# Autodesk Inventor assembly: Draft_02_Combined
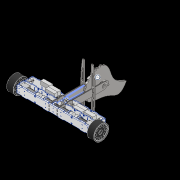
[picture p0: Inventor's stored thumbnail of the model, 180x180]
Saved by Autodesk Inventor 2021 (Build 250183000, 183)
## iProperties
Created: 2021-03-10
Part Number: Draft_02_Combined
Document SubType Name: Assembly
Designer: M3rob
Mass: 102210 g
Surface Area: 54892 cm^2
Volume: 35052.9 cm^3
Density: 2.91588 g/cm^3
Author: M3rob
## Documents named in this file (38)
- C:\Users\Esketitttttt\Documents\GrabCAD\FireBird 250 Pound Gaming Machine\Drafts\FrameDrafts\Draft_Wide01\Draft_Wide01_Combined.iam
- C:\Users\Esketitttttt\Documents\GrabCAD\FireBird 250 Pound Gaming Machine\Drafts\FrameDrafts\Draft_Wide01\NeckFrame_03.ipt
- C:\Users\Esketitttttt\Documents\GrabCAD\FireBird 250 Pound Gaming Machine\Drafts\FrameDrafts\Draft_Wide01\FrontWallFrame_03.ipt
- C:\Users\Esketitttttt\Documents\GrabCAD\FireBird 250 Pound Gaming Machine\Drafts\FrameDrafts\Draft_Wide01\BackWallFrame_03.ipt
- C:\Users\Esketitttttt\Documents\GrabCAD\FireBird 250 Pound Gaming Machine\Drafts\FrameDrafts\Draft_Wide01\SmallSideFrame_03.ipt
- C:\Users\Esketitttttt\Documents\GrabCAD\FireBird 250 Pound Gaming Machine\Drafts\FrameDrafts\Draft_Wide01\DriveSideFrame_03.ipt
- C:\Users\Esketitttttt\Documents\GrabCAD\FireBird 250 Pound Gaming Machine\Drafts\FrameDrafts\Draft_Wide01\6524K421_FRICTION TORQUE LIMITER.ipt
- C:\Users\Esketitttttt\Documents\GrabCAD\FireBird 250 Pound Gaming Machine\Drafts\FrameDrafts\Draft_Wide01\MotorMountingPlates.ipt
- C:\Users\Esketitttttt\Documents\GrabCAD\FireBird 250 Pound Gaming Machine\Drafts\FrameDrafts\Draft_Wide01\MotorMockup.ipt
- C:\Users\Esketitttttt\Documents\GrabCAD\FireBird 250 Pound Gaming Machine\Drafts\FrameDrafts\Draft_Wide01\GearboxMockup.ipt
- C:\Users\M3rob\Documents\Inventor\Content Center Files\R2021\en-US\AS 2465(2)\AS 2465 - 3_8 x 1 1_4  UNC.ipt
- C:\Users\M3rob\Documents\Inventor\Content Center Files\R2021\en-US\AS 2465(1)\AS 2465 - 3_8  UNC(1).ipt
- C:\Users\M3rob\Documents\Inventor\Content Center Files\R2021\en-US\U UNC 2603(1)\Unbrako - 8 x 1 1_4 - 32 - 1.25 - Unbrako.ipt
- C:\Users\M3rob\Documents\Inventor\Content Center Files\R2021\en-US\U UNC 2603(1)\Unbrako - 5_16 x 1 3_4 - 18 - 1.75 - Unbrako.ipt
- C:\Users\Esketitttttt\Documents\GrabCAD\FireBird 250 Pound Gaming Machine\Drafts\FrameDrafts\Draft_Wide01\Chain Drive1.iam
- C:\Users\Esketitttttt\Documents\GrabCAD\FireBird 250 Pound Gaming Machine\Drafts\FrameDrafts\Draft_Wide01\Chain Drive2.iam
- C:\Users\Esketitttttt\Documents\GrabCAD\FireBird 250 Pound Gaming Machine\Drafts\FrameDrafts\Draft_Wide01\Chain Drive3.iam
- C:\Users\Esketitttttt\Documents\GrabCAD\FireBird 250 Pound Gaming Machine\Drafts\FrameDrafts\Draft_Wide01\Bearing1.iam
- C:\Users\Esketitttttt\Documents\GrabCAD\FireBird 250 Pound Gaming Machine\Drafts\FrameDrafts\Draft_Wide01\Shaft4.ipt
- C:\Users\Esketitttttt\Documents\GrabCAD\FireBird 250 Pound Gaming Machine\Drafts\FrameDrafts\Draft_Wide01\WeaponDraft02.ipt
- C:\Users\Esketitttttt\Documents\GrabCAD\FireBird 250 Pound Gaming Machine\Drafts\FrameDrafts\Draft_Wide01\TopBottomUHMW.ipt
- C:\Users\Esketitttttt\Documents\GrabCAD\FireBird 250 Pound Gaming Machine\Drafts\FrameDrafts\Draft_Wide01\FrontWallUHMW.ipt
- C:\Users\Esketitttttt\Documents\GrabCAD\FireBird 250 Pound Gaming Machine\Drafts\FrameDrafts\Draft_Wide01\Bearing3.iam
- C:\Users\Esketitttttt\Documents\GrabCAD\FireBird 250 Pound Gaming Machine\Drafts\FrameDrafts\Draft_Wide01\Shaft5.ipt
- C:\Users\Esketitttttt\Documents\GrabCAD\FireBird 250 Pound Gaming Machine\Drafts\FrameDrafts\Draft_Wide01\SmallFrontWallUHMW.ipt
- C:\Users\M3rob\Documents\Inventor\Content Center Files\R2021\en-US\AS 2465(2)\AS 2465 - 3_8 x 1 1_2  UNC.ipt
- C:\Users\M3rob\Documents\Inventor\Content Center Files\R2021\en-US\ANSI B18.2.2(09)\ANSI B18.2.2 - 3_8 - 16(2).ipt
- C:\Users\M3rob\Documents\Inventor\Content Center Files\R2021\en-US\AS 2465(2)\AS 2465 - 3_8 x 2  UNC.ipt
- C:\Users\M3rob\Documents\Inventor\Content Center Files\R2021\en-US\AS 2465(2)\AS 2465 - 3_8 x 2 1_2  UNC.ipt
- C:\Users\Esketitttttt\Documents\GrabCAD\FireBird 250 Pound Gaming Machine\Drafts\FrameDrafts\Draft_Wide01\MotorCircularClamp.ipt
- C:\Users\Esketitttttt\Documents\GrabCAD\FireBird 250 Pound Gaming Machine\Drafts\FrameDrafts\Draft_Wide01\MotorClampUhmw.ipt
- C:\Users\Esketitttttt\Documents\GrabCAD\FireBird 250 Pound Gaming Machine\Drafts\FrameDrafts\Draft_Wide01\MockupWheel.ipt
- C:\Users\Esketitttttt\Documents\GrabCAD\FireBird 250 Pound Gaming Machine\Drafts\FrameDrafts\Draft_Wide01\WheelHubMockup.ipt
- C:\Users\Esketitttttt\Documents\GrabCAD\FireBird 250 Pound Gaming Machine\Drafts\FrameDrafts\Draft_Wide01\ThiccUpright.ipt
- C:\Users\Esketitttttt\Documents\GrabCAD\FireBird 250 Pound Gaming Machine\Drafts\FrameDrafts\Draft_Wide01\Battery Mockup.ipt
- C:\Users\Esketitttttt\Documents\GrabCAD\FireBird 250 Pound Gaming Machine\Drafts\FrameDrafts\Draft_Wide01\EscMockup.ipt
- C:\Users\Esketitttttt\Documents\GrabCAD\FireBird 250 Pound Gaming Machine\Drafts\FrameDrafts\Draft_Wide01\Whyachi_MS-2PowerSwitch.ipt
- C:\Users\Esketitttttt\Documents\GrabCAD\FireBird 250 Pound Gaming Machine\Drafts\FrameDrafts\Draft_Wide01\MidWallFrame_03.ipt
## Components (214 placed, 33 different names)
1. NeckFrame_03:1 — Mate:1, Mate:3, Mate:4, Mate:5, Mate:12, Mate:14, Mate:17, Mate:18, Mate:40, Mate:41, Mate:42, Mate:47, Mate:71, Mate:73, Mate:75, Mate:77, Mate:98, Mate:99, Mate:104, Flush:4, Mate:125, Flush:18, Mate:260, Mate:384, Mate:385, Mate:386
2. NeckFrame_03:2 — Mate:1, Mate:6, Mate:7, Mate:8, Mate:9, Mate:10, Mate:11, Mate:19, Mate:43, Mate:44, Mate:45, Mate:46, Mate:87, Mate:89, Mate:91, Mate:93, Mate:103, Mate:105, Flush:3, Mate:110, Mate:111, Mate:119, Mate:123, Mate:124, Mate:381, Mate:382, Mate:383, Flush:46, Mate:420
3. MidWallFrame_03:1 — Mate:9, Mate:10, Mate:11, Mate:20, Mate:21, Mate:22
4. FrontWallFrame_03:2 — Mate:6, Mate:7, Mate:8, Flush:10, Flush:11, Mate:165, Mate:167, Mate:169, Mate:171, Mate:173, Mate:175, Mate:177, Mate:179, Mate:181, Mate:183, Mate:185, Mate:187, Mate:189, Mate:191, Mate:193, Mate:195, Mate:229, Mate:231, Mate:233, Mate:235, Mate:237, Mate:239, Mate:241, Mate:243, Mate:245, Mate:247, Mate:249, Mate:251, Mate:253, Mate:255, Mate:257, Mate:259, Mate:276, Mate:278, Mate:280, Mate:282, Mate:284, Mate:286
5. FrontWallFrame_03:3 — Mate:3, Mate:4, Mate:5, Mate:23, Mate:24, Mate:25, Mate:300, Mate:302, Mate:304, Mate:306, Mate:308, Mate:310
6. MidWallFrame_03:2 — Mate:12, Mate:14, Mate:260, Mate:410
7. BackWallFrame_03:1 — Mate:17, Mate:18, Mate:19, Mate:37, Mate:38, Mate:348, Mate:350, Mate:352, Mate:354, Mate:356, Mate:358, Mate:360, Mate:362, Mate:364, Mate:366, Mate:368, Mate:370, Mate:372, Mate:374, Mate:418, Mate:419, Flush:45, Flush:46, Mate:420, Flush:47
8. SmallSideFrame_03:1 — Mate:20, Mate:21, Mate:22, Flush:9, Flush:13, Mate:128
9. SmallSideFrame_03:2 — Mate:23, Mate:24, Mate:25, Mate:261, Mate:316, Mate:318
10. DriveSideFrame_03:1 — Insert:9, Insert:10, Insert:11, Insert:12, Mate:378, Mate:379, Mate:380, Insert:27, Mate:418, Mate:419, Flush:45
11. DriveSideFrame_03:2 — Mate:37, Mate:38, Mate:57, Mate:59, Insert:13, Insert:14, Insert:15, Insert:16, Mate:377, Insert:29, Flush:47
12. 6524K421_FRICTION TORQUE LIMITER:1 — Mate:94, Flush:2, Mate:96
13. 6524K421_FRICTION TORQUE LIMITER:2 — Mate:95, Flush:1, Mate:97
14. Chain Drive:1 [sub-assembly]
15. Chain Drive:2 [sub-assembly] — Mate:112, Mate:375
16. Chain Drive:3 [sub-assembly]
17. Bearing:1 [sub-assembly] — Mate:103, Mate:104
18. Bearing:2 [sub-assembly] — Mate:105, Flush:3
19. Shaft:1 — Mate:112, Mate:113, Angle:1
20. WeaponDraft02:1 — Mate:110, Mate:111
21. TopBottomUHMW:1 — Flush:11, Flush:13, Mate:196, Mate:197, Mate:198, Mate:199, Mate:200, Mate:201, Mate:202, Mate:203, Mate:204, Mate:205, Mate:206, Mate:207, Mate:208, Mate:209, Mate:210, Mate:211, Mate:212, Mate:213, Mate:214, Mate:215, Mate:216, Mate:217, Mate:218, Mate:219, Mate:220, Mate:221, Mate:222, Mate:223, Mate:224, Mate:225, Mate:226, Mate:227, Mate:228, Mate:230, Mate:232, Mate:234, Mate:236, Mate:238, Mate:240, Mate:242, Mate:244, Mate:246, Mate:248, Mate:250, Mate:252, Mate:254, Mate:256, Mate:258
22. TopBottomUHMW:2 — Flush:9, Flush:10, Mate:118, Flush:14, Flush:19, Mate:132, Mate:133, Mate:134, Mate:135, Mate:136, Mate:137, Mate:138, Mate:139, Mate:140, Mate:141, Mate:142, Mate:143, Mate:144, Mate:145, Mate:146, Mate:147, Mate:148, Mate:149, Mate:150, Mate:151, Mate:152, Mate:153, Mate:154, Mate:155, Mate:156, Mate:157, Mate:158, Mate:159, Mate:160, Mate:161, Mate:162, Mate:163, Mate:164, Mate:166, Mate:168, Mate:170, Mate:172, Mate:174, Mate:176, Mate:178, Mate:180, Mate:182, Mate:184, Mate:186, Mate:188, Mate:190, Mate:192, Mate:194, Flush:23
23. FrontWallUHMW:1 — Mate:118, Flush:14, Mate:119, Mate:129, Mate:263, Mate:264, Mate:265, Mate:266, Mate:267, Mate:268, Mate:269, Mate:270, Mate:271, Mate:272, Mate:273, Mate:274, Mate:275, Mate:277, Mate:279, Mate:281, Mate:283, Mate:285
24. Bearing:3 [sub-assembly] — Mate:123, Mate:124
25. SmallFrontWallUHMW:1 — Mate:261, Flush:23, Mate:311, Mate:312, Mate:313, Mate:314, Mate:315, Mate:317
26. SmallFrontWallUHMW:2 — Mate:128, Mate:129, Flush:19
27. ThiccUpright:1 — Mate:381, Mate:382, Mate:383
28. ThiccUpright:2 — Mate:384, Mate:385, Mate:386
29. MotorMountingPlates:1 — Mate:40, Mate:41, Mate:42, Mate:49, Mate:62, Mate:63, Mate:64, Mate:65, Mate:66, Mate:67, Mate:68, Mate:69, Mate:70, Mate:72, Mate:74, Mate:76, Insert:5, Insert:6, Insert:7, Insert:8, Mate:96
30. MotorMountingPlates:2 — Mate:43, Mate:44, Mate:45, Mate:50, Mate:78, Mate:79, Mate:80, Mate:81, Mate:82, Mate:83, Mate:84, Mate:85, Mate:86, Mate:88, Mate:90, Mate:92, Insert:1, Insert:2, Insert:3, Insert:4, Mate:97
31. MotorMockup:1 — Mate:46, Mate:50, Mate:95, Flush:1, Insert:21
32. MotorMockup:2 — Mate:47, Mate:49, Mate:94, Flush:2, Insert:24
33. MotorMockup:3 — Mate:60, Mate:61, Insert:23
34. MotorMockup:4 — Insert:22, Insert:25
35. GearboxMockup:1 — Mate:57, Mate:59, Mate:60, Mate:61, Mate:377, Angle:4
36. GearboxMockup:2 — Mate:378, Mate:379, Mate:380, Insert:25, Angle:3
37. AS 2465 - Inch 3/8 x 1 1/4  UNC:1 — Mate:62, Mate:63
38. AS 2465 - Inch 3/8  UNC:1 — Mate:70, Mate:71
39. AS 2465 - Inch 3/8 x 1 1/4  UNC:2 — Mate:64, Mate:65
40. AS 2465 - Inch 3/8 x 1 1/4  UNC:3 — Mate:66, Mate:67
41. AS 2465 - Inch 3/8 x 1 1/4  UNC:4 — Mate:68, Mate:69
42. AS 2465 - Inch 3/8  UNC:2 — Mate:72, Mate:73
43. AS 2465 - Inch 3/8  UNC:3 — Mate:74, Mate:75
44. AS 2465 - Inch 3/8  UNC:4 — Mate:76, Mate:77
45. AS 2465 - Inch 3/8 x 1 1/4  UNC:5 — Mate:78, Mate:79
46. AS 2465 - Inch 3/8  UNC:5 — Mate:86, Mate:87
47. AS 2465 - Inch 3/8 x 1 1/4  UNC:6 — Mate:80, Mate:81
48. AS 2465 - Inch 3/8 x 1 1/4  UNC:7 — Mate:82, Mate:83
49. AS 2465 - Inch 3/8 x 1 1/4  UNC:8 — Mate:84, Mate:85
50. AS 2465 - Inch 3/8  UNC:6 — Mate:88, Mate:89
51. AS 2465 - Inch 3/8  UNC:7 — Mate:90, Mate:91
52. AS 2465 - Inch 3/8  UNC:8 — Mate:92, Mate:93
53. Unbrako UNC Hex Socket Cap - Inch 8 x 1 1/4:1 — Insert:1
54. Unbrako UNC Hex Socket Cap - Inch 8 x 1 1/4:2 — Insert:2
55. Unbrako UNC Hex Socket Cap - Inch 8 x 1 1/4:3 — Insert:3
56. Unbrako UNC Hex Socket Cap - Inch 8 x 1 1/4:4 — Insert:4
57. Unbrako UNC Hex Socket Cap - Inch 8 x 1 1/4:5 — Insert:5
58. Unbrako UNC Hex Socket Cap - Inch 8 x 1 1/4:6 — Insert:6
59. Unbrako UNC Hex Socket Cap - Inch 8 x 1 1/4:7 — Insert:7
60. Unbrako UNC Hex Socket Cap - Inch 8 x 1 1/4:8 — Insert:8
61. Unbrako UNC Hex Socket Cap - Inch 5/16 x 1 3/4:1 — Insert:9
62. Unbrako UNC Hex Socket Cap - Inch 5/16 x 1 3/4:2 — Insert:10
63. Unbrako UNC Hex Socket Cap - Inch 5/16 x 1 3/4:3 — Insert:11
64. Unbrako UNC Hex Socket Cap - Inch 5/16 x 1 3/4:4 — Insert:12
65. Unbrako UNC Hex Socket Cap - Inch 5/16 x 1 3/4:5 — Insert:13
66. Unbrako UNC Hex Socket Cap - Inch 5/16 x 1 3/4:6 — Insert:14
67. Unbrako UNC Hex Socket Cap - Inch 5/16 x 1 3/4:7 — Insert:15
68. Unbrako UNC Hex Socket Cap - Inch 5/16 x 1 3/4:8 — Insert:16
69. Bearing:4 [sub-assembly] — Mate:125, Flush:18
70. Shaft:1 — Mate:375, Mate:376, Angle:2
71. AS 2465 - Inch 3/8 x 1 1/2  UNC:1 — Mate:132, Mate:133
72. Hex Nut - Inch 3/8 - 16:1 — Mate:164, Mate:165
73. AS 2465 - Inch 3/8 x 1 1/2  UNC:2 — Mate:134, Mate:135
74. AS 2465 - Inch 3/8 x 1 1/2  UNC:3 — Mate:136, Mate:137
75. AS 2465 - Inch 3/8 x 1 1/2  UNC:4 — Mate:138, Mate:139
76. AS 2465 - Inch 3/8 x 1 1/2  UNC:5 — Mate:140, Mate:141
77. AS 2465 - Inch 3/8 x 1 1/2  UNC:6 — Mate:142, Mate:143
78. AS 2465 - Inch 3/8 x 1 1/2  UNC:7 — Mate:144, Mate:145
79. AS 2465 - Inch 3/8 x 1 1/2  UNC:8 — Mate:146, Mate:147
80. AS 2465 - Inch 3/8 x 1 1/2  UNC:9 — Mate:148, Mate:149
81. AS 2465 - Inch 3/8 x 1 1/2  UNC:10 — Mate:150, Mate:151
82. AS 2465 - Inch 3/8 x 1 1/2  UNC:11 — Mate:152, Mate:153
83. AS 2465 - Inch 3/8 x 1 1/2  UNC:12 — Mate:154, Mate:155
84. AS 2465 - Inch 3/8 x 1 1/2  UNC:13 — Mate:156, Mate:157
85. AS 2465 - Inch 3/8 x 1 1/2  UNC:14 — Mate:158, Mate:159
86. AS 2465 - Inch 3/8 x 1 1/2  UNC:15 — Mate:160, Mate:161
87. AS 2465 - Inch 3/8 x 1 1/2  UNC:16 — Mate:162, Mate:163
88. Hex Nut - Inch 3/8 - 16:2 — Mate:166, Mate:167
89. Hex Nut - Inch 3/8 - 16:3 — Mate:168, Mate:169
90. Hex Nut - Inch 3/8 - 16:4 — Mate:170, Mate:171
91. Hex Nut - Inch 3/8 - 16:5 — Mate:172, Mate:173
92. Hex Nut - Inch 3/8 - 16:6 — Mate:174, Mate:175
93. Hex Nut - Inch 3/8 - 16:7 — Mate:176, Mate:177
94. Hex Nut - Inch 3/8 - 16:8 — Mate:178, Mate:179
95. Hex Nut - Inch 3/8 - 16:9 — Mate:180, Mate:181
96. Hex Nut - Inch 3/8 - 16:10 — Mate:182, Mate:183
97. Hex Nut - Inch 3/8 - 16:11 — Mate:184, Mate:185
98. Hex Nut - Inch 3/8 - 16:12 — Mate:186, Mate:187
99. Hex Nut - Inch 3/8 - 16:13 — Mate:188, Mate:189
100. Hex Nut - Inch 3/8 - 16:14 — Mate:190, Mate:191
101. Hex Nut - Inch 3/8 - 16:15 — Mate:192, Mate:193
102. Hex Nut - Inch 3/8 - 16:16 — Mate:194, Mate:195
103. AS 2465 - Inch 3/8 x 1 1/2  UNC:17 — Mate:196, Mate:197
104. Hex Nut - Inch 3/8 - 16:17 — Mate:228, Mate:229
105. AS 2465 - Inch 3/8 x 1 1/2  UNC:18 — Mate:198, Mate:199
106. AS 2465 - Inch 3/8 x 1 1/2  UNC:19 — Mate:200, Mate:201
107. AS 2465 - Inch 3/8 x 1 1/2  UNC:20 — Mate:202, Mate:203
108. AS 2465 - Inch 3/8 x 1 1/2  UNC:21 — Mate:204, Mate:205
109. AS 2465 - Inch 3/8 x 1 1/2  UNC:22 — Mate:206, Mate:207
110. AS 2465 - Inch 3/8 x 1 1/2  UNC:23 — Mate:208, Mate:209
111. AS 2465 - Inch 3/8 x 1 1/2  UNC:24 — Mate:210, Mate:211
112. AS 2465 - Inch 3/8 x 1 1/2  UNC:25 — Mate:212, Mate:213
113. AS 2465 - Inch 3/8 x 1 1/2  UNC:26 — Mate:214, Mate:215
114. AS 2465 - Inch 3/8 x 1 1/2  UNC:27 — Mate:216, Mate:217
115. AS 2465 - Inch 3/8 x 1 1/2  UNC:28 — Mate:218, Mate:219
116. AS 2465 - Inch 3/8 x 1 1/2  UNC:29 — Mate:220, Mate:221
117. AS 2465 - Inch 3/8 x 1 1/2  UNC:30 — Mate:222, Mate:223
118. AS 2465 - Inch 3/8 x 1 1/2  UNC:31 — Mate:224, Mate:225
119. AS 2465 - Inch 3/8 x 1 1/2  UNC:32 — Mate:226, Mate:227
120. Hex Nut - Inch 3/8 - 16:18 — Mate:230, Mate:231
121. Hex Nut - Inch 3/8 - 16:19 — Mate:232, Mate:233
122. Hex Nut - Inch 3/8 - 16:20 — Mate:234, Mate:235
123. Hex Nut - Inch 3/8 - 16:21 — Mate:236, Mate:237
124. Hex Nut - Inch 3/8 - 16:22 — Mate:238, Mate:239
125. Hex Nut - Inch 3/8 - 16:23 — Mate:240, Mate:241
126. Hex Nut - Inch 3/8 - 16:24 — Mate:242, Mate:243
127. Hex Nut - Inch 3/8 - 16:25 — Mate:244, Mate:245
128. Hex Nut - Inch 3/8 - 16:26 — Mate:246, Mate:247
129. Hex Nut - Inch 3/8 - 16:27 — Mate:248, Mate:249
130. Hex Nut - Inch 3/8 - 16:28 — Mate:250, Mate:251
131. Hex Nut - Inch 3/8 - 16:29 — Mate:252, Mate:253
132. Hex Nut - Inch 3/8 - 16:30 — Mate:254, Mate:255
133. Hex Nut - Inch 3/8 - 16:31 — Mate:256, Mate:257
134. Hex Nut - Inch 3/8 - 16:32 — Mate:258, Mate:259
135. AS 2465 - Inch 3/8 x 2  UNC:1 — Mate:263, Mate:264
136. AS 2465 - Inch 3/8  UNC:9 — Mate:275, Mate:276
137. AS 2465 - Inch 3/8 x 2  UNC:2 — Mate:265, Mate:266
138. AS 2465 - Inch 3/8 x 2  UNC:3 — Mate:267, Mate:268
139. AS 2465 - Inch 3/8 x 2  UNC:4 — Mate:269, Mate:270
140. AS 2465 - Inch 3/8 x 2  UNC:5 — Mate:271, Mate:272
141. AS 2465 - Inch 3/8 x 2  UNC:6 — Mate:273, Mate:274
142. AS 2465 - Inch 3/8  UNC:10 — Mate:277, Mate:278
143. AS 2465 - Inch 3/8  UNC:11 — Mate:279, Mate:280
144. AS 2465 - Inch 3/8  UNC:12 — Mate:281, Mate:282
145. AS 2465 - Inch 3/8  UNC:13 — Mate:283, Mate:284
146. AS 2465 - Inch 3/8  UNC:14 — Mate:285, Mate:286
147. AS 2465 - Inch 3/8 x 2  UNC:7
148. AS 2465 - Inch 3/8  UNC:15 — Mate:300
149. AS 2465 - Inch 3/8 x 2  UNC:8
150. AS 2465 - Inch 3/8 x 2  UNC:9
151. AS 2465 - Inch 3/8 x 2  UNC:10
152. AS 2465 - Inch 3/8 x 2  UNC:11
153. AS 2465 - Inch 3/8 x 2  UNC:12
154. AS 2465 - Inch 3/8  UNC:16 — Mate:302
155. AS 2465 - Inch 3/8  UNC:17 — Mate:304
156. AS 2465 - Inch 3/8  UNC:18 — Mate:306
157. AS 2465 - Inch 3/8  UNC:19 — Mate:308
158. AS 2465 - Inch 3/8  UNC:20 — Mate:310
159. AS 2465 - Inch 3/8 x 2  UNC:13 — Mate:311, Mate:312
160. AS 2465 - Inch 3/8  UNC:21 — Mate:315, Mate:316
161. AS 2465 - Inch 3/8 x 2  UNC:14 — Mate:313, Mate:314
162. AS 2465 - Inch 3/8  UNC:22 — Mate:317, Mate:318
163. AS 2465 - Inch 3/8 x 2 1/2  UNC:1
164. AS 2465 - Inch 3/8  UNC:23 — Mate:348
165. AS 2465 - Inch 3/8 x 2 1/2  UNC:2
166. AS 2465 - Inch 3/8 x 2 1/2  UNC:3
167. AS 2465 - Inch 3/8 x 2 1/2  UNC:4
168. AS 2465 - Inch 3/8 x 2 1/2  UNC:5
169. AS 2465 - Inch 3/8 x 2 1/2  UNC:6
170. AS 2465 - Inch 3/8 x 2 1/2  UNC:7
171. AS 2465 - Inch 3/8 x 2 1/2  UNC:8
172. AS 2465 - Inch 3/8 x 2 1/2  UNC:9
173. AS 2465 - Inch 3/8 x 2 1/2  UNC:10
174. AS 2465 - Inch 3/8 x 2 1/2  UNC:11
175. AS 2465 - Inch 3/8 x 2 1/2  UNC:12
176. AS 2465 - Inch 3/8 x 2 1/2  UNC:13
177. AS 2465 - Inch 3/8 x 2 1/2  UNC:14
178. AS 2465 - Inch 3/8  UNC:24 — Mate:350
179. AS 2465 - Inch 3/8  UNC:25 — Mate:352
180. AS 2465 - Inch 3/8  UNC:26 — Mate:354
181. AS 2465 - Inch 3/8  UNC:27 — Mate:356
182. AS 2465 - Inch 3/8  UNC:28 — Mate:358
183. AS 2465 - Inch 3/8  UNC:29 — Mate:360
184. AS 2465 - Inch 3/8  UNC:30 — Mate:362
185. AS 2465 - Inch 3/8  UNC:31 — Mate:364
186. AS 2465 - Inch 3/8  UNC:32 — Mate:366
187. AS 2465 - Inch 3/8  UNC:33 — Mate:368
188. AS 2465 - Inch 3/8  UNC:34 — Mate:370
189. AS 2465 - Inch 3/8  UNC:35 — Mate:372
190. AS 2465 - Inch 3/8  UNC:36 — Mate:374
191. MockupWheel:1 — Insert:26
192. MockupWheel:2 — Insert:28
193. WheelHubMockup:1 — Insert:28, Insert:29, Angle:4
194. WheelHubMockup:2 — Insert:26, Insert:27, Angle:3
195. Whyachi_MS-2PowerSwitch:2
196. Whyachi_MS-2PowerSwitch:1
197. EscMockup:1
198. EscMockup:2 — Mate:406
199. EscMockup:3 — Mate:409
200. EscMockup:4
201. Battery Mockup:1 — Mate:390, Flush:28, Flush:32, Mate:406
202. Battery Mockup:2 — Mate:390, Flush:28, Flush:32, Mate:407, Flush:33
203. Battery Mockup:3 — Mate:407, Flush:33
204. Battery Mockup:4 — Mate:388, Flush:24, Flush:31, Mate:410
205. Battery Mockup:5 — Mate:388, Flush:24, Flush:31, Mate:408, Flush:34, Mate:409
206. Battery Mockup:6 — Mate:408, Flush:34
207. MotorCircularClamp:1 — Insert:19
208. MotorClampUhmw:1 — Insert:19, Insert:22
209. MotorCircularClamp:2 — Insert:20
210. MotorClampUhmw:2 — Insert:20, Insert:21
211. MotorCircularClamp:3 — Insert:18
212. MotorClampUhmw:3 — Insert:18, Insert:24
213. MotorCircularClamp:4 — Insert:17
214. MotorClampUhmw:4 — Insert:17, Insert:23
## Relationships (351: Mate 297, Insert 29, Flush 21, Angle 4)
- Mate:1: NeckFrame_03:1 ↔ NeckFrame_03:2
- Mate:3: NeckFrame_03:1 ↔ FrontWallFrame_03:3
- Mate:4: NeckFrame_03:1 ↔ FrontWallFrame_03:3
- Mate:5: NeckFrame_03:1 ↔ FrontWallFrame_03:3
- Mate:6: NeckFrame_03:2 ↔ FrontWallFrame_03:2
- Mate:7: NeckFrame_03:2 ↔ FrontWallFrame_03:2
- Mate:8: NeckFrame_03:2 ↔ FrontWallFrame_03:2
- Mate:9: NeckFrame_03:2 ↔ MidWallFrame_03:1
- Mate:10: NeckFrame_03:2 ↔ MidWallFrame_03:1
- Mate:11: NeckFrame_03:2 ↔ MidWallFrame_03:1
- Mate:12: NeckFrame_03:1 ↔ MidWallFrame_03:2
- Mate:14: NeckFrame_03:1 ↔ MidWallFrame_03:2
- Mate:17: NeckFrame_03:1 ↔ BackWallFrame_03:1
- Mate:18: NeckFrame_03:1 ↔ BackWallFrame_03:1
- Mate:19: NeckFrame_03:2 ↔ BackWallFrame_03:1
- Mate:20: MidWallFrame_03:1 ↔ SmallSideFrame_03:1
- Mate:21: MidWallFrame_03:1 ↔ SmallSideFrame_03:1
- Mate:22: MidWallFrame_03:1 ↔ SmallSideFrame_03:1
- Mate:23: FrontWallFrame_03:3 ↔ SmallSideFrame_03:2
- Mate:24: FrontWallFrame_03:3 ↔ SmallSideFrame_03:2
- Mate:25: FrontWallFrame_03:3 ↔ SmallSideFrame_03:2
- Mate:37: BackWallFrame_03:1 ↔ DriveSideFrame_03:2
- Mate:38: BackWallFrame_03:1 ↔ DriveSideFrame_03:2
- Mate:40: NeckFrame_03:1 ↔ MotorMountingPlates:1
- Mate:41: NeckFrame_03:1 ↔ MotorMountingPlates:1
- Mate:42: NeckFrame_03:1 ↔ MotorMountingPlates:1
- Mate:43: NeckFrame_03:2 ↔ MotorMountingPlates:2
- Mate:44: NeckFrame_03:2 ↔ MotorMountingPlates:2
- Mate:45: NeckFrame_03:2 ↔ MotorMountingPlates:2
- Mate:46: NeckFrame_03:2 ↔ MotorMockup:1
- Mate:47: NeckFrame_03:1 ↔ MotorMockup:2
- Mate:49: MotorMountingPlates:1 ↔ MotorMockup:2
- Mate:50: MotorMountingPlates:2 ↔ MotorMockup:1
- Mate:57: DriveSideFrame_03:2 ↔ GearboxMockup:1
- Mate:59: DriveSideFrame_03:2 ↔ GearboxMockup:1
- Mate:60: MotorMockup:3 ↔ GearboxMockup:1
- Mate:61: MotorMockup:3 ↔ GearboxMockup:1
- Mate:62: MotorMountingPlates:1 ↔ AS 2465 - Inch 3/8 x 1 1/4  UNC:1
- Mate:63: MotorMountingPlates:1 ↔ AS 2465 - Inch 3/8 x 1 1/4  UNC:1
- Mate:64: MotorMountingPlates:1 ↔ AS 2465 - Inch 3/8 x 1 1/4  UNC:2
- Mate:65: MotorMountingPlates:1 ↔ AS 2465 - Inch 3/8 x 1 1/4  UNC:2
- Mate:66: MotorMountingPlates:1 ↔ AS 2465 - Inch 3/8 x 1 1/4  UNC:3
- Mate:67: MotorMountingPlates:1 ↔ AS 2465 - Inch 3/8 x 1 1/4  UNC:3
- Mate:68: MotorMountingPlates:1 ↔ AS 2465 - Inch 3/8 x 1 1/4  UNC:4
- Mate:69: MotorMountingPlates:1 ↔ AS 2465 - Inch 3/8 x 1 1/4  UNC:4
- Mate:70: MotorMountingPlates:1 ↔ AS 2465 - Inch 3/8  UNC:1
- Mate:71: NeckFrame_03:1 ↔ AS 2465 - Inch 3/8  UNC:1
- Mate:72: MotorMountingPlates:1 ↔ AS 2465 - Inch 3/8  UNC:2
- Mate:73: NeckFrame_03:1 ↔ AS 2465 - Inch 3/8  UNC:2
- Mate:74: MotorMountingPlates:1 ↔ AS 2465 - Inch 3/8  UNC:3
- Mate:75: NeckFrame_03:1 ↔ AS 2465 - Inch 3/8  UNC:3
- Mate:76: MotorMountingPlates:1 ↔ AS 2465 - Inch 3/8  UNC:4
- Mate:77: NeckFrame_03:1 ↔ AS 2465 - Inch 3/8  UNC:4
- Mate:78: MotorMountingPlates:2 ↔ AS 2465 - Inch 3/8 x 1 1/4  UNC:5
- Mate:79: MotorMountingPlates:2 ↔ AS 2465 - Inch 3/8 x 1 1/4  UNC:5
- Mate:80: MotorMountingPlates:2 ↔ AS 2465 - Inch 3/8 x 1 1/4  UNC:6
- Mate:81: MotorMountingPlates:2 ↔ AS 2465 - Inch 3/8 x 1 1/4  UNC:6
- Mate:82: MotorMountingPlates:2 ↔ AS 2465 - Inch 3/8 x 1 1/4  UNC:7
- Mate:83: MotorMountingPlates:2 ↔ AS 2465 - Inch 3/8 x 1 1/4  UNC:7
- Mate:84: MotorMountingPlates:2 ↔ AS 2465 - Inch 3/8 x 1 1/4  UNC:8
- Mate:85: MotorMountingPlates:2 ↔ AS 2465 - Inch 3/8 x 1 1/4  UNC:8
- Mate:86: MotorMountingPlates:2 ↔ AS 2465 - Inch 3/8  UNC:5
- Mate:87: NeckFrame_03:2 ↔ AS 2465 - Inch 3/8  UNC:5
- Mate:88: MotorMountingPlates:2 ↔ AS 2465 - Inch 3/8  UNC:6
- Mate:89: NeckFrame_03:2 ↔ AS 2465 - Inch 3/8  UNC:6
- Mate:90: MotorMountingPlates:2 ↔ AS 2465 - Inch 3/8  UNC:7
- Mate:91: NeckFrame_03:2 ↔ AS 2465 - Inch 3/8  UNC:7
- Mate:92: MotorMountingPlates:2 ↔ AS 2465 - Inch 3/8  UNC:8
- Mate:93: NeckFrame_03:2 ↔ AS 2465 - Inch 3/8  UNC:8
- Insert:1: MotorMountingPlates:2 ↔ Unbrako UNC Hex Socket Cap - Inch 8 x 1 1/4:1
- Insert:2: MotorMountingPlates:2 ↔ Unbrako UNC Hex Socket Cap - Inch 8 x 1 1/4:2
- Insert:3: MotorMountingPlates:2 ↔ Unbrako UNC Hex Socket Cap - Inch 8 x 1 1/4:3
- Insert:4: MotorMountingPlates:2 ↔ Unbrako UNC Hex Socket Cap - Inch 8 x 1 1/4:4
- Insert:5: MotorMountingPlates:1 ↔ Unbrako UNC Hex Socket Cap - Inch 8 x 1 1/4:5
- Insert:6: MotorMountingPlates:1 ↔ Unbrako UNC Hex Socket Cap - Inch 8 x 1 1/4:6
- Insert:7: MotorMountingPlates:1 ↔ Unbrako UNC Hex Socket Cap - Inch 8 x 1 1/4:7
- Insert:8: MotorMountingPlates:1 ↔ Unbrako UNC Hex Socket Cap - Inch 8 x 1 1/4:8
- Insert:9: DriveSideFrame_03:1 ↔ Unbrako UNC Hex Socket Cap - Inch 5/16 x 1 3/4:1
- Insert:10: DriveSideFrame_03:1 ↔ Unbrako UNC Hex Socket Cap - Inch 5/16 x 1 3/4:2
- Insert:11: DriveSideFrame_03:1 ↔ Unbrako UNC Hex Socket Cap - Inch 5/16 x 1 3/4:3
- Insert:12: DriveSideFrame_03:1 ↔ Unbrako UNC Hex Socket Cap - Inch 5/16 x 1 3/4:4
- Insert:13: DriveSideFrame_03:2 ↔ Unbrako UNC Hex Socket Cap - Inch 5/16 x 1 3/4:5
- Insert:14: DriveSideFrame_03:2 ↔ Unbrako UNC Hex Socket Cap - Inch 5/16 x 1 3/4:6
- Insert:15: DriveSideFrame_03:2 ↔ Unbrako UNC Hex Socket Cap - Inch 5/16 x 1 3/4:7
- Insert:16: DriveSideFrame_03:2 ↔ Unbrako UNC Hex Socket Cap - Inch 5/16 x 1 3/4:8
- Mate:94: 6524K421_FRICTION TORQUE LIMITER:1 ↔ MotorMockup:2
- Mate:95: 6524K421_FRICTION TORQUE LIMITER:2 ↔ MotorMockup:1
- Flush:1: 6524K421_FRICTION TORQUE LIMITER:2 ↔ MotorMockup:1
- Flush:2: 6524K421_FRICTION TORQUE LIMITER:1 ↔ MotorMockup:2
- Mate:96 (1.5875 mm): 6524K421_FRICTION TORQUE LIMITER:1 ↔ MotorMountingPlates:1
- Mate:97 (1.5875 mm): 6524K421_FRICTION TORQUE LIMITER:2 ↔ MotorMountingPlates:2
- Mate:98: NeckFrame_03:1
- Mate:99: NeckFrame_03:1
- Mate:100
- Mate:101
- Mate:103: NeckFrame_03:2 ↔ Bearing:1
- Mate:104: NeckFrame_03:1 ↔ Bearing:1
- Mate:105: NeckFrame_03:2 ↔ Bearing:2
- Flush:3: NeckFrame_03:2 ↔ Bearing:2
- Flush:4 (19.05 mm): NeckFrame_03:1
- Mate:108
- Mate:109
- Mate:110: NeckFrame_03:2 ↔ WeaponDraft02:1
- Mate:111 (25.4 mm): NeckFrame_03:2 ↔ WeaponDraft02:1
- Mate:112: Chain Drive:2 ↔ Shaft:1
- Mate:113: Shaft:1
- Angle:1 (0 deg): Shaft:1
- Flush:9: SmallSideFrame_03:1 ↔ TopBottomUHMW:2
- Flush:10: FrontWallFrame_03:2 ↔ TopBottomUHMW:2
- Flush:11: FrontWallFrame_03:2 ↔ TopBottomUHMW:1
- Flush:13: SmallSideFrame_03:1 ↔ TopBottomUHMW:1
- Mate:118: TopBottomUHMW:2 ↔ FrontWallUHMW:1
- Flush:14: TopBottomUHMW:2 ↔ FrontWallUHMW:1
- Mate:119: NeckFrame_03:2 ↔ FrontWallUHMW:1
- Mate:123: NeckFrame_03:2 ↔ Bearing:3
- Mate:124: NeckFrame_03:2 ↔ Bearing:3
- Mate:125: NeckFrame_03:1 ↔ Bearing:4
- Flush:18: NeckFrame_03:1 ↔ Bearing:4
- Mate:128: SmallSideFrame_03:1 ↔ SmallFrontWallUHMW:2
- Mate:129: FrontWallUHMW:1 ↔ SmallFrontWallUHMW:2
- Flush:19: TopBottomUHMW:2 ↔ SmallFrontWallUHMW:2
- Mate:132: TopBottomUHMW:2 ↔ AS 2465 - Inch 3/8 x 1 1/2  UNC:1
- Mate:133: TopBottomUHMW:2 ↔ AS 2465 - Inch 3/8 x 1 1/2  UNC:1
- Mate:134: TopBottomUHMW:2 ↔ AS 2465 - Inch 3/8 x 1 1/2  UNC:2
- Mate:135: TopBottomUHMW:2 ↔ AS 2465 - Inch 3/8 x 1 1/2  UNC:2
- Mate:136: TopBottomUHMW:2 ↔ AS 2465 - Inch 3/8 x 1 1/2  UNC:3
- Mate:137: TopBottomUHMW:2 ↔ AS 2465 - Inch 3/8 x 1 1/2  UNC:3
- Mate:138: TopBottomUHMW:2 ↔ AS 2465 - Inch 3/8 x 1 1/2  UNC:4
- Mate:139: TopBottomUHMW:2 ↔ AS 2465 - Inch 3/8 x 1 1/2  UNC:4
- Mate:140: TopBottomUHMW:2 ↔ AS 2465 - Inch 3/8 x 1 1/2  UNC:5
- Mate:141: TopBottomUHMW:2 ↔ AS 2465 - Inch 3/8 x 1 1/2  UNC:5
- Mate:142: TopBottomUHMW:2 ↔ AS 2465 - Inch 3/8 x 1 1/2  UNC:6
- Mate:143: TopBottomUHMW:2 ↔ AS 2465 - Inch 3/8 x 1 1/2  UNC:6
- Mate:144: TopBottomUHMW:2 ↔ AS 2465 - Inch 3/8 x 1 1/2  UNC:7
- Mate:145: TopBottomUHMW:2 ↔ AS 2465 - Inch 3/8 x 1 1/2  UNC:7
- Mate:146: TopBottomUHMW:2 ↔ AS 2465 - Inch 3/8 x 1 1/2  UNC:8
- Mate:147: TopBottomUHMW:2 ↔ AS 2465 - Inch 3/8 x 1 1/2  UNC:8
- Mate:148: TopBottomUHMW:2 ↔ AS 2465 - Inch 3/8 x 1 1/2  UNC:9
- Mate:149: TopBottomUHMW:2 ↔ AS 2465 - Inch 3/8 x 1 1/2  UNC:9
- Mate:150: TopBottomUHMW:2 ↔ AS 2465 - Inch 3/8 x 1 1/2  UNC:10
- Mate:151: TopBottomUHMW:2 ↔ AS 2465 - Inch 3/8 x 1 1/2  UNC:10
- Mate:152: TopBottomUHMW:2 ↔ AS 2465 - Inch 3/8 x 1 1/2  UNC:11
- Mate:153: TopBottomUHMW:2 ↔ AS 2465 - Inch 3/8 x 1 1/2  UNC:11
- Mate:154: TopBottomUHMW:2 ↔ AS 2465 - Inch 3/8 x 1 1/2  UNC:12
- Mate:155: TopBottomUHMW:2 ↔ AS 2465 - Inch 3/8 x 1 1/2  UNC:12
- Mate:156: TopBottomUHMW:2 ↔ AS 2465 - Inch 3/8 x 1 1/2  UNC:13
- Mate:157: TopBottomUHMW:2 ↔ AS 2465 - Inch 3/8 x 1 1/2  UNC:13
- Mate:158: TopBottomUHMW:2 ↔ AS 2465 - Inch 3/8 x 1 1/2  UNC:14
- Mate:159: TopBottomUHMW:2 ↔ AS 2465 - Inch 3/8 x 1 1/2  UNC:14
- Mate:160: TopBottomUHMW:2 ↔ AS 2465 - Inch 3/8 x 1 1/2  UNC:15
- Mate:161: TopBottomUHMW:2 ↔ AS 2465 - Inch 3/8 x 1 1/2  UNC:15
- Mate:162: TopBottomUHMW:2 ↔ AS 2465 - Inch 3/8 x 1 1/2  UNC:16
- Mate:163: TopBottomUHMW:2 ↔ AS 2465 - Inch 3/8 x 1 1/2  UNC:16
- Mate:164: TopBottomUHMW:2 ↔ Hex Nut - Inch 3/8 - 16:1
- Mate:165: FrontWallFrame_03:2 ↔ Hex Nut - Inch 3/8 - 16:1
- Mate:166: TopBottomUHMW:2 ↔ Hex Nut - Inch 3/8 - 16:2
- Mate:167: FrontWallFrame_03:2 ↔ Hex Nut - Inch 3/8 - 16:2
- Mate:168: TopBottomUHMW:2 ↔ Hex Nut - Inch 3/8 - 16:3
- Mate:169: FrontWallFrame_03:2 ↔ Hex Nut - Inch 3/8 - 16:3
- Mate:170: TopBottomUHMW:2 ↔ Hex Nut - Inch 3/8 - 16:4
- Mate:171: FrontWallFrame_03:2 ↔ Hex Nut - Inch 3/8 - 16:4
- Mate:172: TopBottomUHMW:2 ↔ Hex Nut - Inch 3/8 - 16:5
- Mate:173: FrontWallFrame_03:2 ↔ Hex Nut - Inch 3/8 - 16:5
- Mate:174: TopBottomUHMW:2 ↔ Hex Nut - Inch 3/8 - 16:6
- Mate:175: FrontWallFrame_03:2 ↔ Hex Nut - Inch 3/8 - 16:6
- Mate:176: TopBottomUHMW:2 ↔ Hex Nut - Inch 3/8 - 16:7
- Mate:177: FrontWallFrame_03:2 ↔ Hex Nut - Inch 3/8 - 16:7
- Mate:178: TopBottomUHMW:2 ↔ Hex Nut - Inch 3/8 - 16:8
- Mate:179: FrontWallFrame_03:2 ↔ Hex Nut - Inch 3/8 - 16:8
- Mate:180: TopBottomUHMW:2 ↔ Hex Nut - Inch 3/8 - 16:9
- Mate:181: FrontWallFrame_03:2 ↔ Hex Nut - Inch 3/8 - 16:9
- Mate:182: TopBottomUHMW:2 ↔ Hex Nut - Inch 3/8 - 16:10
- Mate:183: FrontWallFrame_03:2 ↔ Hex Nut - Inch 3/8 - 16:10
- Mate:184: TopBottomUHMW:2 ↔ Hex Nut - Inch 3/8 - 16:11
- Mate:185: FrontWallFrame_03:2 ↔ Hex Nut - Inch 3/8 - 16:11
- Mate:186: TopBottomUHMW:2 ↔ Hex Nut - Inch 3/8 - 16:12
- Mate:187: FrontWallFrame_03:2 ↔ Hex Nut - Inch 3/8 - 16:12
- Mate:188: TopBottomUHMW:2 ↔ Hex Nut - Inch 3/8 - 16:13
- Mate:189: FrontWallFrame_03:2 ↔ Hex Nut - Inch 3/8 - 16:13
- Mate:190: TopBottomUHMW:2 ↔ Hex Nut - Inch 3/8 - 16:14
- Mate:191: FrontWallFrame_03:2 ↔ Hex Nut - Inch 3/8 - 16:14
- Mate:192: TopBottomUHMW:2 ↔ Hex Nut - Inch 3/8 - 16:15
- Mate:193: FrontWallFrame_03:2 ↔ Hex Nut - Inch 3/8 - 16:15
- Mate:194: TopBottomUHMW:2 ↔ Hex Nut - Inch 3/8 - 16:16
- Mate:195: FrontWallFrame_03:2 ↔ Hex Nut - Inch 3/8 - 16:16
- Mate:196: TopBottomUHMW:1 ↔ AS 2465 - Inch 3/8 x 1 1/2  UNC:17
- Mate:197: TopBottomUHMW:1 ↔ AS 2465 - Inch 3/8 x 1 1/2  UNC:17
- Mate:198: TopBottomUHMW:1 ↔ AS 2465 - Inch 3/8 x 1 1/2  UNC:18
- Mate:199: TopBottomUHMW:1 ↔ AS 2465 - Inch 3/8 x 1 1/2  UNC:18
- Mate:200: TopBottomUHMW:1 ↔ AS 2465 - Inch 3/8 x 1 1/2  UNC:19
- Mate:201: TopBottomUHMW:1 ↔ AS 2465 - Inch 3/8 x 1 1/2  UNC:19
- Mate:202: TopBottomUHMW:1 ↔ AS 2465 - Inch 3/8 x 1 1/2  UNC:20
- Mate:203: TopBottomUHMW:1 ↔ AS 2465 - Inch 3/8 x 1 1/2  UNC:20
- Mate:204: TopBottomUHMW:1 ↔ AS 2465 - Inch 3/8 x 1 1/2  UNC:21
- Mate:205: TopBottomUHMW:1 ↔ AS 2465 - Inch 3/8 x 1 1/2  UNC:21
- Mate:206: TopBottomUHMW:1 ↔ AS 2465 - Inch 3/8 x 1 1/2  UNC:22
- Mate:207: TopBottomUHMW:1 ↔ AS 2465 - Inch 3/8 x 1 1/2  UNC:22
- Mate:208: TopBottomUHMW:1 ↔ AS 2465 - Inch 3/8 x 1 1/2  UNC:23
- Mate:209: TopBottomUHMW:1 ↔ AS 2465 - Inch 3/8 x 1 1/2  UNC:23
- Mate:210: TopBottomUHMW:1 ↔ AS 2465 - Inch 3/8 x 1 1/2  UNC:24
- Mate:211: TopBottomUHMW:1 ↔ AS 2465 - Inch 3/8 x 1 1/2  UNC:24
- Mate:212: TopBottomUHMW:1 ↔ AS 2465 - Inch 3/8 x 1 1/2  UNC:25
- Mate:213: TopBottomUHMW:1 ↔ AS 2465 - Inch 3/8 x 1 1/2  UNC:25
- Mate:214: TopBottomUHMW:1 ↔ AS 2465 - Inch 3/8 x 1 1/2  UNC:26
- Mate:215: TopBottomUHMW:1 ↔ AS 2465 - Inch 3/8 x 1 1/2  UNC:26
- Mate:216: TopBottomUHMW:1 ↔ AS 2465 - Inch 3/8 x 1 1/2  UNC:27
- Mate:217: TopBottomUHMW:1 ↔ AS 2465 - Inch 3/8 x 1 1/2  UNC:27
- Mate:218: TopBottomUHMW:1 ↔ AS 2465 - Inch 3/8 x 1 1/2  UNC:28
- Mate:219: TopBottomUHMW:1 ↔ AS 2465 - Inch 3/8 x 1 1/2  UNC:28
- Mate:220: TopBottomUHMW:1 ↔ AS 2465 - Inch 3/8 x 1 1/2  UNC:29
- Mate:221: TopBottomUHMW:1 ↔ AS 2465 - Inch 3/8 x 1 1/2  UNC:29
- Mate:222: TopBottomUHMW:1 ↔ AS 2465 - Inch 3/8 x 1 1/2  UNC:30
- Mate:223: TopBottomUHMW:1 ↔ AS 2465 - Inch 3/8 x 1 1/2  UNC:30
- Mate:224: TopBottomUHMW:1 ↔ AS 2465 - Inch 3/8 x 1 1/2  UNC:31
- Mate:225: TopBottomUHMW:1 ↔ AS 2465 - Inch 3/8 x 1 1/2  UNC:31
- Mate:226: TopBottomUHMW:1 ↔ AS 2465 - Inch 3/8 x 1 1/2  UNC:32
- Mate:227: TopBottomUHMW:1 ↔ AS 2465 - Inch 3/8 x 1 1/2  UNC:32
- Mate:228: TopBottomUHMW:1 ↔ Hex Nut - Inch 3/8 - 16:17
- Mate:229: FrontWallFrame_03:2 ↔ Hex Nut - Inch 3/8 - 16:17
- Mate:230: TopBottomUHMW:1 ↔ Hex Nut - Inch 3/8 - 16:18
- Mate:231: FrontWallFrame_03:2 ↔ Hex Nut - Inch 3/8 - 16:18
- Mate:232: TopBottomUHMW:1 ↔ Hex Nut - Inch 3/8 - 16:19
- Mate:233: FrontWallFrame_03:2 ↔ Hex Nut - Inch 3/8 - 16:19
- Mate:234: TopBottomUHMW:1 ↔ Hex Nut - Inch 3/8 - 16:20
- Mate:235: FrontWallFrame_03:2 ↔ Hex Nut - Inch 3/8 - 16:20
- Mate:236: TopBottomUHMW:1 ↔ Hex Nut - Inch 3/8 - 16:21
- Mate:237: FrontWallFrame_03:2 ↔ Hex Nut - Inch 3/8 - 16:21
- Mate:238: TopBottomUHMW:1 ↔ Hex Nut - Inch 3/8 - 16:22
- Mate:239: FrontWallFrame_03:2 ↔ Hex Nut - Inch 3/8 - 16:22
- Mate:240: TopBottomUHMW:1 ↔ Hex Nut - Inch 3/8 - 16:23
- Mate:241: FrontWallFrame_03:2 ↔ Hex Nut - Inch 3/8 - 16:23
- Mate:242: TopBottomUHMW:1 ↔ Hex Nut - Inch 3/8 - 16:24
- Mate:243: FrontWallFrame_03:2 ↔ Hex Nut - Inch 3/8 - 16:24
- Mate:244: TopBottomUHMW:1 ↔ Hex Nut - Inch 3/8 - 16:25
- Mate:245: FrontWallFrame_03:2 ↔ Hex Nut - Inch 3/8 - 16:25
- Mate:246: TopBottomUHMW:1 ↔ Hex Nut - Inch 3/8 - 16:26
- Mate:247: FrontWallFrame_03:2 ↔ Hex Nut - Inch 3/8 - 16:26
- Mate:248: TopBottomUHMW:1 ↔ Hex Nut - Inch 3/8 - 16:27
- Mate:249: FrontWallFrame_03:2 ↔ Hex Nut - Inch 3/8 - 16:27
- Mate:250: TopBottomUHMW:1 ↔ Hex Nut - Inch 3/8 - 16:28
- Mate:251: FrontWallFrame_03:2 ↔ Hex Nut - Inch 3/8 - 16:28
- Mate:252: TopBottomUHMW:1 ↔ Hex Nut - Inch 3/8 - 16:29
- Mate:253: FrontWallFrame_03:2 ↔ Hex Nut - Inch 3/8 - 16:29
- Mate:254: TopBottomUHMW:1 ↔ Hex Nut - Inch 3/8 - 16:30
- Mate:255: FrontWallFrame_03:2 ↔ Hex Nut - Inch 3/8 - 16:30
- Mate:256: TopBottomUHMW:1 ↔ Hex Nut - Inch 3/8 - 16:31
- Mate:257: FrontWallFrame_03:2 ↔ Hex Nut - Inch 3/8 - 16:31
- Mate:258: TopBottomUHMW:1 ↔ Hex Nut - Inch 3/8 - 16:32
- Mate:259: FrontWallFrame_03:2 ↔ Hex Nut - Inch 3/8 - 16:32
- Mate:260: NeckFrame_03:1 ↔ MidWallFrame_03:2
- Mate:261: SmallSideFrame_03:2 ↔ SmallFrontWallUHMW:1
- Flush:23: TopBottomUHMW:2 ↔ SmallFrontWallUHMW:1
- Mate:263: FrontWallUHMW:1 ↔ AS 2465 - Inch 3/8 x 2  UNC:1
- Mate:264: FrontWallUHMW:1 ↔ AS 2465 - Inch 3/8 x 2  UNC:1
- Mate:265: FrontWallUHMW:1 ↔ AS 2465 - Inch 3/8 x 2  UNC:2
- Mate:266: FrontWallUHMW:1 ↔ AS 2465 - Inch 3/8 x 2  UNC:2
- Mate:267: FrontWallUHMW:1 ↔ AS 2465 - Inch 3/8 x 2  UNC:3
- Mate:268: FrontWallUHMW:1 ↔ AS 2465 - Inch 3/8 x 2  UNC:3
- Mate:269: FrontWallUHMW:1 ↔ AS 2465 - Inch 3/8 x 2  UNC:4
- Mate:270: FrontWallUHMW:1 ↔ AS 2465 - Inch 3/8 x 2  UNC:4
- Mate:271: FrontWallUHMW:1 ↔ AS 2465 - Inch 3/8 x 2  UNC:5
- Mate:272: FrontWallUHMW:1 ↔ AS 2465 - Inch 3/8 x 2  UNC:5
- Mate:273: FrontWallUHMW:1 ↔ AS 2465 - Inch 3/8 x 2  UNC:6
- Mate:274: FrontWallUHMW:1 ↔ AS 2465 - Inch 3/8 x 2  UNC:6
- Mate:275: FrontWallUHMW:1 ↔ AS 2465 - Inch 3/8  UNC:9
- Mate:276: FrontWallFrame_03:2 ↔ AS 2465 - Inch 3/8  UNC:9
- Mate:277: FrontWallUHMW:1 ↔ AS 2465 - Inch 3/8  UNC:10
- Mate:278: FrontWallFrame_03:2 ↔ AS 2465 - Inch 3/8  UNC:10
- Mate:279: FrontWallUHMW:1 ↔ AS 2465 - Inch 3/8  UNC:11
- Mate:280: FrontWallFrame_03:2 ↔ AS 2465 - Inch 3/8  UNC:11
- Mate:281: FrontWallUHMW:1 ↔ AS 2465 - Inch 3/8  UNC:12
- Mate:282: FrontWallFrame_03:2 ↔ AS 2465 - Inch 3/8  UNC:12
- Mate:283: FrontWallUHMW:1 ↔ AS 2465 - Inch 3/8  UNC:13
- Mate:284: FrontWallFrame_03:2 ↔ AS 2465 - Inch 3/8  UNC:13
- Mate:285: FrontWallUHMW:1 ↔ AS 2465 - Inch 3/8  UNC:14
- Mate:286: FrontWallFrame_03:2 ↔ AS 2465 - Inch 3/8  UNC:14
- Mate:300: FrontWallFrame_03:3 ↔ AS 2465 - Inch 3/8  UNC:15
- Mate:302: FrontWallFrame_03:3 ↔ AS 2465 - Inch 3/8  UNC:16
- Mate:304: FrontWallFrame_03:3 ↔ AS 2465 - Inch 3/8  UNC:17
- Mate:306: FrontWallFrame_03:3 ↔ AS 2465 - Inch 3/8  UNC:18
- Mate:308: FrontWallFrame_03:3 ↔ AS 2465 - Inch 3/8  UNC:19
- Mate:310: FrontWallFrame_03:3 ↔ AS 2465 - Inch 3/8  UNC:20
- Mate:311: SmallFrontWallUHMW:1 ↔ AS 2465 - Inch 3/8 x 2  UNC:13
- Mate:312: SmallFrontWallUHMW:1 ↔ AS 2465 - Inch 3/8 x 2  UNC:13
- Mate:313: SmallFrontWallUHMW:1 ↔ AS 2465 - Inch 3/8 x 2  UNC:14
- Mate:314: SmallFrontWallUHMW:1 ↔ AS 2465 - Inch 3/8 x 2  UNC:14
- Mate:315: SmallFrontWallUHMW:1 ↔ AS 2465 - Inch 3/8  UNC:21
- Mate:316: SmallSideFrame_03:2 ↔ AS 2465 - Inch 3/8  UNC:21
- Mate:317: SmallFrontWallUHMW:1 ↔ AS 2465 - Inch 3/8  UNC:22
- Mate:318: SmallSideFrame_03:2 ↔ AS 2465 - Inch 3/8  UNC:22
- Mate:348: BackWallFrame_03:1 ↔ AS 2465 - Inch 3/8  UNC:23
- Mate:350: BackWallFrame_03:1 ↔ AS 2465 - Inch 3/8  UNC:24
- Mate:352: BackWallFrame_03:1 ↔ AS 2465 - Inch 3/8  UNC:25
- Mate:354: BackWallFrame_03:1 ↔ AS 2465 - Inch 3/8  UNC:26
- Mate:356: BackWallFrame_03:1 ↔ AS 2465 - Inch 3/8  UNC:27
- Mate:358: BackWallFrame_03:1 ↔ AS 2465 - Inch 3/8  UNC:28
- Mate:360: BackWallFrame_03:1 ↔ AS 2465 - Inch 3/8  UNC:29
- Mate:362: BackWallFrame_03:1 ↔ AS 2465 - Inch 3/8  UNC:30
- Mate:364: BackWallFrame_03:1 ↔ AS 2465 - Inch 3/8  UNC:31
- Mate:366: BackWallFrame_03:1 ↔ AS 2465 - Inch 3/8  UNC:32
- Mate:368: BackWallFrame_03:1 ↔ AS 2465 - Inch 3/8  UNC:33
- Mate:370: BackWallFrame_03:1 ↔ AS 2465 - Inch 3/8  UNC:34
- Mate:372: BackWallFrame_03:1 ↔ AS 2465 - Inch 3/8  UNC:35
- Mate:374: BackWallFrame_03:1 ↔ AS 2465 - Inch 3/8  UNC:36
- Mate:375: Chain Drive:2 ↔ Shaft:1
- Mate:376: Shaft:1
- Angle:2 (0 deg): Shaft:1
- Insert:17: MotorCircularClamp:4 ↔ MotorClampUhmw:4
- Insert:18: MotorCircularClamp:3 ↔ MotorClampUhmw:3
- Insert:19: MotorCircularClamp:1 ↔ MotorClampUhmw:1
- Insert:20: MotorCircularClamp:2 ↔ MotorClampUhmw:2
- Insert:21 (12.7 mm): MotorMockup:1 ↔ MotorClampUhmw:2
- Insert:22 (12.7 mm): MotorMockup:4 ↔ MotorClampUhmw:1
- Insert:23 (12.7 mm): MotorMockup:3 ↔ MotorClampUhmw:4
- Insert:24 (12.7 mm): MotorMockup:2 ↔ MotorClampUhmw:3
- Mate:377: DriveSideFrame_03:2 ↔ GearboxMockup:1
- Mate:378: DriveSideFrame_03:1 ↔ GearboxMockup:2
- Mate:379: DriveSideFrame_03:1 ↔ GearboxMockup:2
- Mate:380: DriveSideFrame_03:1 ↔ GearboxMockup:2
- Insert:25: MotorMockup:4 ↔ GearboxMockup:2
- Mate:381: NeckFrame_03:2 ↔ ThiccUpright:1
- Mate:382: NeckFrame_03:2 ↔ ThiccUpright:1
- Mate:383: NeckFrame_03:2 ↔ ThiccUpright:1
- Mate:384: NeckFrame_03:1 ↔ ThiccUpright:2
- Mate:385: NeckFrame_03:1 ↔ ThiccUpright:2
- Mate:386: NeckFrame_03:1 ↔ ThiccUpright:2
- Mate:388: Battery Mockup:4 ↔ Battery Mockup:5
- Flush:24: Battery Mockup:4 ↔ Battery Mockup:5
- Mate:390: Battery Mockup:1 ↔ Battery Mockup:2
- Flush:28: Battery Mockup:1 ↔ Battery Mockup:2
- Flush:31: Battery Mockup:4 ↔ Battery Mockup:5
- Insert:26 (-6.35 mm): MockupWheel:1 ↔ WheelHubMockup:2
- Insert:27: DriveSideFrame_03:1 ↔ WheelHubMockup:2
- Angle:3 (0 deg): GearboxMockup:2 ↔ WheelHubMockup:2
- Insert:28 (-6.35 mm): MockupWheel:2 ↔ WheelHubMockup:1
- Insert:29: DriveSideFrame_03:2 ↔ WheelHubMockup:1
- Angle:4 (0 deg): GearboxMockup:1 ↔ WheelHubMockup:1
- Flush:32: Battery Mockup:1 ↔ Battery Mockup:2
- Mate:406 (6.35 mm): EscMockup:2 ↔ Battery Mockup:1
- Mate:407: Battery Mockup:2 ↔ Battery Mockup:3
- Flush:33: Battery Mockup:2 ↔ Battery Mockup:3
- Mate:408: Battery Mockup:5 ↔ Battery Mockup:6
- Flush:34: Battery Mockup:5 ↔ Battery Mockup:6
- Mate:409 (6.35 mm): EscMockup:3 ↔ Battery Mockup:5
- Mate:410: MidWallFrame_03:2 ↔ Battery Mockup:4
- Mate:418: BackWallFrame_03:1 ↔ DriveSideFrame_03:1
- Mate:419: BackWallFrame_03:1 ↔ DriveSideFrame_03:1
- Flush:45: BackWallFrame_03:1 ↔ DriveSideFrame_03:1
- Flush:46: NeckFrame_03:2 ↔ BackWallFrame_03:1
- Mate:420: NeckFrame_03:2 ↔ BackWallFrame_03:1
- Flush:47: BackWallFrame_03:1 ↔ DriveSideFrame_03:2
